# Autodesk Inventor assembly: ASSEMBLY PISTON
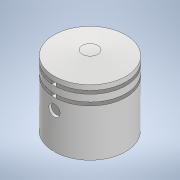
[picture p0: Inventor's stored thumbnail of the model, 180x180]
Saved by Autodesk Inventor 2020 (Build 240168000, 168)
## iProperties
Created: 2021-07-04
Part Number: ASSEMBLY PISTON
Document SubType Name: Assembly
Designer: lokes
Author: lokes
## Documents named in this file (4)
- C:\Users\lokes\OneDrive\Desktop\major\ASSEMBLY PISTON.iam
- C:\Users\lokes\OneDrive\Desktop\major\PISTON.ipt
- C:\Users\lokes\OneDrive\Desktop\major\PISTON COMPRESSION RING.ipt
- C:\Users\lokes\OneDrive\Documents\Inventor\Content Center Files\R2020\en-US\ISO 2338(2)\ISO 2338 - 5 h8 x 30.ipt
## Components (4 placed, 3 different names)
1. PISTON:1 — Mate:1, Mate:2, Mate:3, Mate:4, Mate:5, Mate:6, Mate:8
2. PISTON COMPRESSION RING:1 — Mate:4, Mate:5, Mate:7
3. PISTON COMPRESSION RING:2 — Mate:1, Mate:2, Mate:3, Mate:6, Mate:7
4. ISO 2338 5 h8 x 30:1 — Mate:8
## Relationships (8: Mate 8)
- Mate:1: PISTON:1 ↔ PISTON COMPRESSION RING:2
- Mate:2: PISTON:1 ↔ PISTON COMPRESSION RING:2
- Mate:3: PISTON:1 ↔ PISTON COMPRESSION RING:2
- Mate:4: PISTON:1 ↔ PISTON COMPRESSION RING:1
- Mate:5: PISTON:1 ↔ PISTON COMPRESSION RING:1
- Mate:6: PISTON:1 ↔ PISTON COMPRESSION RING:2
- Mate:7: PISTON COMPRESSION RING:1 ↔ PISTON COMPRESSION RING:2
- Mate:8: PISTON:1 ↔ ISO 2338 5 h8 x 30:1
